# Autodesk Inventor assembly: Telescope
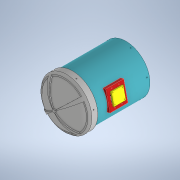
[picture p0: Inventor's stored thumbnail of the model, 180x180]
Saved by Autodesk Inventor 2022 (Build 260153000, 153)
## iProperties
Created: 2023-08-20
Part Number: Telescope
Document SubType Name: Assembly
Designer: fouad
Author: fouad
## Documents named in this file (8)
- C:\Users\fouad\Documents\Telescope\Telescope.iam
- C:\Users\fouad\Documents\Telescope\Aperture.ipt
- C:\Users\fouad\Documents\Telescope\Main Mirror, f=24mm.ipt
- C:\Users\fouad\Documents\Telescope\Viewing Mirror.ipt
- C:\Users\fouad\Documents\Telescope\Viewing Mirror Holder.ipt
- C:\Users\fouad\Documents\Telescope\Viewing Mirror Holder Mount.ipt
- C:\Users\fouad\Documents\Telescope\Eyepiece Mount.ipt
- C:\Users\fouad\Documents\Telescope\Lens Holder.ipt
## Components (8 placed, 7 different names)
1. Main Mirror, f=24mm:1
2. Viewing Mirror:1 — Rigid:1
3. Aperture:1 — Angle:1, Mate:2, Mate:4, Mate:5, Tangent:2, Mate:6, Tangent:3, Mate:7, Angle:2, Mate:8, Rigid:2, Rigid:3
4. Viewing Mirror Holder:1 — Flush:1, Flush:2, Flush:3, Mate:2, Symmetry:1, Rigid:1
5. Viewing Mirror Holder Mount:1 — Flush:1, Flush:2, Flush:3, Angle:1, Mate:4
6. Eyepiece Mount:1 — Mate:7, Angle:2, Mate:8, Mate:9, Flush:5, Flush:6
7. Lens Holder:1 — Mate:9, Flush:5, Flush:6, Symmetry:1
8. Main Mirror, f=24mm:2 — Rigid:2, Rigid:3
## Relationships (20: Mate 7, Flush 5, WeldJoint 3, Angle 2, Tangent 2, Symmetry 1)
- Flush:1 (3 mm): Viewing Mirror Holder:1 ↔ Viewing Mirror Holder Mount:1
- Flush:2 (-1 mm): Viewing Mirror Holder:1 ↔ Viewing Mirror Holder Mount:1
- Flush:3 (3 mm): Viewing Mirror Holder:1 ↔ Viewing Mirror Holder Mount:1
- Angle:1 (0 deg): Aperture:1 ↔ Viewing Mirror Holder Mount:1
- Mate:2 (1.5 mm): Aperture:1 ↔ Viewing Mirror Holder:1
- Mate:4 (-2.55 mm): Aperture:1 ↔ Viewing Mirror Holder Mount:1
- Mate:5: Aperture:1
- Tangent:2: Aperture:1
- Mate:6: Aperture:1
- Tangent:3: Aperture:1
- Mate:7 (-1.5 mm): Aperture:1 ↔ Eyepiece Mount:1
- Angle:2 (0 deg): Aperture:1 ↔ Eyepiece Mount:1
- Mate:8 (-3 mm): Aperture:1 ↔ Eyepiece Mount:1
- Mate:9: Eyepiece Mount:1 ↔ Lens Holder:1
- Flush:5: Eyepiece Mount:1 ↔ Lens Holder:1
- Flush:6 (2 mm): Eyepiece Mount:1 ↔ Lens Holder:1
- Symmetry:1: Viewing Mirror Holder:1 ↔ Lens Holder:1
- Rigid:1 [WeldJoint]: Viewing Mirror:1 ↔ Viewing Mirror Holder:1
- Rigid:2 [WeldJoint]: Aperture:1 ↔ Main Mirror, f=24mm:2
- Rigid:3 [WeldJoint]: Aperture:1 ↔ Main Mirror, f=24mm:2
